# Autodesk Inventor assembly: OsnovanieWood
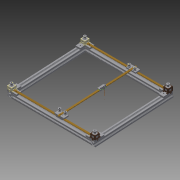
[picture p0: Inventor's stored thumbnail of the model, 180x180]
Saved by Autodesk Inventor 2015 (Build 190159000, 159)
## iProperties
Created: 2016-04-26
Part Number: OsnovanieWood
Document SubType Name: Assembly
Designer: Andreas
Author: Andreas
## Documents named in this file (16)
- C:\Users\criit\Desktop\проект\ласт_ворк_v1.5.1\OsnovanieWood.iam
- C:\Users\criit\Desktop\проект\ласт_ворк_v1.5.1\Balka.ipt
- C:\Users\criit\Desktop\проект\ласт_ворк_v1.5.1\wooden1.ipt
- C:\Users\criit\Desktop\проект\ласт_ворк_v1.5.1\relsa2.ipt
- C:\Users\criit\Desktop\проект\ласт_ворк_v1.5.1\левая каретка+деталь к ней\Сборка.iam
- C:\Users\criit\Desktop\проект\ласт_ворк_v1.5.1\Katushka.ipt
- C:\Users\criit\Desktop\проект\ласт_ворк_v1.5.1\shtuka_ot_motorchika2015.ipt
- C:\Users\criit\Desktop\проект\ласт_ворк_v1.5.1\Motor.ipt
- C:\Users\criit\Desktop\проект\ласт_ворк_v1.5.1\laser.ipt
- C:\Users\criit\Desktop\проект\ласт_ворк_v1.5.1\ray.ipt
- C:\Users\criit\Desktop\проект\ласт_ворк_v1.5.1\новая каретка\Karetka.ipt
- C:\Users\criit\Desktop\проект\ласт_ворк_v1.5.1\Podshipnik.ipt
- C:\Users\criit\Desktop\проект\ласт_ворк_v1.5.1\ygolki.ipt
- C:\Users\criit\Desktop\проект\ласт_ворк_v1.5.1\dop_krepl_k_sponke_ne_motora.ipt
- C:\Users\criit\Desktop\проект\ласт_ворк_v1.5.1\zaporkaShponki.ipt
- C:\Users\criit\Desktop\проект\ласт_ворк_v1.5.1\клешня под шпоньку\kleshnya.ipt
## Components (50 placed, 15 different names)
1. Balka:1 — Rigid:1, Rigid:2, Mate:1, Flush:1, Flush:2, Mate:62, Flush:36, Flush:37
2. Balka:2 — Rigid:1, Rigid:3
3. Balka:3 — Rigid:3, Flush:5, Flush:6, Mate:3, Mate:65, Flush:41, Flush:42
4. Balka:4 — Rigid:2
5. wooden1:1 — Mate:1, Flush:1, Flush:2, Flush:9, Mate:34, Flush:34, Flush:35, Mate:53
6. wooden1:2 — Mate:62, Flush:36, Flush:37, Mate:63, Flush:38, Flush:39, Mate:64, Mate:67, Flush:45
7. wooden1:3 — Flush:5, Flush:6, Mate:3, Mate:5, Flush:10, Mate:87, Mate:90, Flush:52, Flush:53
8. wooden1:4 — Mate:65, Flush:41, Flush:42, Mate:86, Mate:91, Flush:54, Flush:55
9. relsa2:1 — Mate:5, Flush:9, Flush:10, Mate:7, Mate:8
10. relsa2:2 — Mate:67, Flush:45, Mate:68, Mate:69, Mate:70
11. Сборка:1 [sub-assembly] — Mate:7, Mate:8, Flush:22, Flush:23, Mate:22, Flush:24, Mate:26, Mate:27, Mate:31, Mate:32, Mate:47, Mate:48, Mate:80, Tangent:17, Mate:81, Tangent:18
12. relsa2:3 — Flush:23, Mate:22, Flush:24, Mate:24, Mate:25
13. Katushka:2 — Mate:30, Rotational:9, Rotational:15, Mate:49
14. Katushka:3 — Tangent:7, Flush:46, Flush:47, Tangent:8
15. Katushka:5 — Mate:26, Mate:31, Rotational:7, Rotational:13, Mate:48
16. Katushka:6 — Mate:27, Mate:32, Rotational:6, Rotational:12, Mate:47
17. Katushka:11 — Cylindrical:19, Rotational:8, Rotational:14, Mate:50
18. Katushka:12 — Tangent:10, Mate:73, Mate:74, Tangent:11
19. shtuka_ot_motorchika2015:1 — Mate:43, Mate:44
20. shtuka_ot_motorchika2015:2 — Mate:41, Mate:42
21. Motor:1 — Mate:38, Mate:40, Mate:41, Mate:42, Mate:64
22. Motor:2 — Mate:43, Mate:44, Mate:51, Mate:52, Mate:53
23. laser:1 — Rigid:18, Rigid:19
24. ray:1 — Rigid:18
25. Сборка:2 [sub-assembly] — Flush:22, Cylindrical:19, Mate:30, Mate:49, Mate:50, Mate:69, Mate:70, Mate:78, Tangent:15, Mate:79, Tangent:16
26. Karetka:2 — Mate:24, Mate:25, Rigid:19
27. Podshipnik:1 — Mate:74, Tangent:11, Mate:75, Tangent:12
28. Podshipnik:2 — Rotational:14
29. Podshipnik:3 — Flush:47, Tangent:8, Mate:71
30. Podshipnik:4 — Rotational:13
31. Podshipnik:5 — Rotational:6
32. Podshipnik:7 — Rotational:12
33. Podshipnik:8 — Rotational:15
34. Podshipnik:9 — Tangent:10, Mate:73
35. Podshipnik:10 — Rotational:9
36. Podshipnik:11 — Tangent:7, Flush:46, Tangent:9
37. Podshipnik:12 — Rotational:7
38. Podshipnik:13 — Rotational:8
39. ygolki:1 — Mate:38, Mate:40, Mate:63, Flush:38, Flush:39, Mate:68
40. ygolki:2 — Mate:34, Flush:34, Flush:35, Mate:51, Mate:52
41. dop_krepl_k_sponke_ne_motora:1 — Tangent:9, Mate:71, Mate:76, Tangent:13, Mate:86, Mate:92, Mate:93
42. dop_krepl_k_sponke_ne_motora:2 — Mate:75, Tangent:12, Mate:77, Tangent:14, Mate:87, Mate:94, Mate:95
43. zaporkaShponki:1 — Mate:79, Tangent:16
44. zaporkaShponki:2 — Mate:76, Tangent:13
45. zaporkaShponki:3 — Mate:78, Tangent:15
46. zaporkaShponki:5 — Mate:77, Tangent:14
47. zaporkaShponki:6 — Mate:80, Tangent:17
48. zaporkaShponki:7 — Mate:81, Tangent:18
49. kleshnya:1 — Mate:91, Flush:54, Flush:55, Mate:92, Mate:93
50. kleshnya:2 — Mate:90, Flush:52, Flush:53, Mate:94, Mate:95
## Relationships (103: Mate 53, Flush 24, Tangent 12, RevoluteJoint 8, WeldJoint 5, CylindricalJoint 1)
- Rigid:1 [WeldJoint]: Balka:1 ↔ Balka:2
- Rigid:2 [WeldJoint]: Balka:1 ↔ Balka:4
- Rigid:3 [WeldJoint]: Balka:2 ↔ Balka:3
- Mate:1: Balka:1 ↔ wooden1:1
- Flush:1: Balka:1 ↔ wooden1:1
- Flush:2: Balka:1 ↔ wooden1:1
- Flush:5: Balka:3 ↔ wooden1:3
- Flush:6: Balka:3 ↔ wooden1:3
- Mate:3: Balka:3 ↔ wooden1:3
- Mate:5: wooden1:3 ↔ relsa2:1
- Flush:9 (-10 mm): wooden1:1 ↔ relsa2:1
- Flush:10 (30 mm): wooden1:3 ↔ relsa2:1
- Mate:7: relsa2:1 ↔ Сборка:1
- Mate:8: relsa2:1 ↔ Сборка:1
- Rigid:18 [WeldJoint]: laser:1 ↔ ray:1
- Flush:22: Сборка:1 ↔ Сборка:2
- Flush:23 (-5 mm): Сборка:1 ↔ relsa2:3
- Mate:22: Сборка:1 ↔ relsa2:3
- Flush:24 (25 mm): Сборка:1 ↔ relsa2:3
- Mate:24: relsa2:3 ↔ Karetka:2
- Mate:25: relsa2:3 ↔ Karetka:2
- Mate:26: Сборка:1 ↔ Katushka:5
- Mate:27: Сборка:1 ↔ Katushka:6
- Cylindrical:19: Katushka:11 ↔ Сборка:2
- Mate:30: Katushka:2 ↔ Сборка:2
- Mate:31: Сборка:1 ↔ Katushka:5
- Mate:32: Сборка:1 ↔ Katushka:6
- Rotational:6 [RevoluteJoint]: Katushka:6 ↔ Podshipnik:5
- Rotational:7 [RevoluteJoint]: Katushka:5 ↔ Podshipnik:12
- Rotational:8 [RevoluteJoint]: Katushka:11 ↔ Podshipnik:13
- Rotational:9 [RevoluteJoint]: Katushka:2 ↔ Podshipnik:10
- Rotational:12 [RevoluteJoint]: Katushka:6 ↔ Podshipnik:7
- Rotational:13 [RevoluteJoint]: Katushka:5 ↔ Podshipnik:4
- Rotational:14 [RevoluteJoint]: Katushka:11 ↔ Podshipnik:2
- Rotational:15 [RevoluteJoint]: Katushka:2 ↔ Podshipnik:8
- Mate:34: wooden1:1 ↔ ygolki:2
- Mate:38: Motor:1 ↔ ygolki:1
- Mate:40: Motor:1 ↔ ygolki:1
- Mate:41: shtuka_ot_motorchika2015:2 ↔ Motor:1
- Mate:42: shtuka_ot_motorchika2015:2 ↔ Motor:1
- Mate:43: shtuka_ot_motorchika2015:1 ↔ Motor:2
- Mate:44: shtuka_ot_motorchika2015:1 ↔ Motor:2
- Rigid:19 [WeldJoint]: laser:1 ↔ Karetka:2
- Mate:47: Сборка:1 ↔ Katushka:6
- Mate:48: Сборка:1 ↔ Katushka:5
- Mate:49: Katushka:2 ↔ Сборка:2
- Mate:50: Katushka:11 ↔ Сборка:2
- Flush:34: wooden1:1 ↔ ygolki:2
- Flush:35: wooden1:1 ↔ ygolki:2
- Mate:51: Motor:2 ↔ ygolki:2
- Mate:52: Motor:2 ↔ ygolki:2
- Mate:53: wooden1:1 ↔ Motor:2
- Mate:62: Balka:1 ↔ wooden1:2
- Flush:36: Balka:1 ↔ wooden1:2
- Flush:37: Balka:1 ↔ wooden1:2
- Mate:63: wooden1:2 ↔ ygolki:1
- Flush:38: wooden1:2 ↔ ygolki:1
- Flush:39: wooden1:2 ↔ ygolki:1
- Mate:64: wooden1:2 ↔ Motor:1
- Mate:65: Balka:3 ↔ wooden1:4
- Flush:41: Balka:3 ↔ wooden1:4
- Flush:42: Balka:3 ↔ wooden1:4
- Mate:67: wooden1:2 ↔ relsa2:2
- Flush:45 (10 mm): wooden1:2 ↔ relsa2:2
- Mate:68: relsa2:2 ↔ ygolki:1
- Mate:69: relsa2:2 ↔ Сборка:2
- Mate:70: relsa2:2 ↔ Сборка:2
- Tangent:7: Katushka:3 ↔ Podshipnik:11
- Flush:46: Katushka:3 ↔ Podshipnik:11
- Flush:47: Katushka:3 ↔ Podshipnik:3
- Tangent:8: Katushka:3 ↔ Podshipnik:3
- Tangent:9: Podshipnik:11 ↔ dop_krepl_k_sponke_ne_motora:1
- Mate:71: Podshipnik:3 ↔ dop_krepl_k_sponke_ne_motora:1
- Tangent:10: Katushka:12 ↔ Podshipnik:9
- Mate:73: Katushka:12 ↔ Podshipnik:9
- Mate:74: Katushka:12 ↔ Podshipnik:1
- Tangent:11: Katushka:12 ↔ Podshipnik:1
- Mate:75: Podshipnik:1 ↔ dop_krepl_k_sponke_ne_motora:2
- Tangent:12: Podshipnik:1 ↔ dop_krepl_k_sponke_ne_motora:2
- Mate:76: dop_krepl_k_sponke_ne_motora:1 ↔ zaporkaShponki:2
- Tangent:13: dop_krepl_k_sponke_ne_motora:1 ↔ zaporkaShponki:2
- Mate:77: dop_krepl_k_sponke_ne_motora:2 ↔ zaporkaShponki:5
- Tangent:14: dop_krepl_k_sponke_ne_motora:2 ↔ zaporkaShponki:5
- Mate:78: Сборка:2 ↔ zaporkaShponki:3
- Tangent:15: Сборка:2 ↔ zaporkaShponki:3
- Mate:79: Сборка:2 ↔ zaporkaShponki:1
- Tangent:16: Сборка:2 ↔ zaporkaShponki:1
- Mate:80: Сборка:1 ↔ zaporkaShponki:6
- Tangent:17: Сборка:1 ↔ zaporkaShponki:6
- Mate:81: Сборка:1 ↔ zaporkaShponki:7
- Tangent:18: Сборка:1 ↔ zaporkaShponki:7
- Mate:86: wooden1:4 ↔ dop_krepl_k_sponke_ne_motora:1
- Mate:87: wooden1:3 ↔ dop_krepl_k_sponke_ne_motora:2
- Mate:90: wooden1:3 ↔ kleshnya:2
- Flush:52: wooden1:3 ↔ kleshnya:2
- Flush:53: wooden1:3 ↔ kleshnya:2
- Mate:91: wooden1:4 ↔ kleshnya:1
- Flush:54: wooden1:4 ↔ kleshnya:1
- Flush:55: wooden1:4 ↔ kleshnya:1
- Mate:92: dop_krepl_k_sponke_ne_motora:1 ↔ kleshnya:1
- Mate:93: dop_krepl_k_sponke_ne_motora:1 ↔ kleshnya:1
- Mate:94: dop_krepl_k_sponke_ne_motora:2 ↔ kleshnya:2
- Mate:95: dop_krepl_k_sponke_ne_motora:2 ↔ kleshnya:2
